# Autodesk Inventor assembly: SPE48V1 Roldana Acrilico
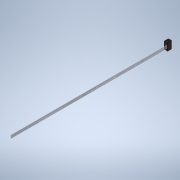
[picture p0: Inventor's stored thumbnail of the model, 180x180]
Saved by Autodesk Inventor 2021.2 (Build 252289000, 289)
## iProperties
Created: 2026-09-01
Part Number: SPE48V1 Roldana Acrilico
Document SubType Name: Assembly
Designer: nelso
Author: nelso
## Documents named in this file (6)
- C:\Users\nelso\Documents\Escritorio\Soporte-Paciente-Espinografia\Workspace\SPE48V1 Roldana Acrilico.iam
- C:\Users\nelso\Documents\Escritorio\Soporte-Paciente-Espinografia\Workspace\SP45V1 Plastico Roldana.ipt
- C:\Users\nelso\Documents\Escritorio\Soporte-Paciente-Espinografia\Workspace\SP46V1 Felpa Roldana.ipt
- C:\Users\nelso\Documents\Escritorio\Soporte-Paciente-Espinografia\Workspace\SP50V1 Acrilico Roldana.ipt
- C:\Users\nelso\Documents\Escritorio\Soporte-Paciente-Espinografia\Workspace\DIN963M3X0.5L10C.ipt
- C:\Users\nelso\Documents\Escritorio\Soporte-Paciente-Espinografia\Workspace\DIN555-5M3X0.5I.ipt
## Components (8 placed, 5 different names)
1. SP45V1 Plastico Roldana:1 — Mate:1, Mate:2, Flush:1, Flush:2, Flush:3, Mate:3, Mate:4, Mate:5, Mate:6, Mate:11, Mate:12
2. SP46V1 Felpa Roldana:1 — Mate:1, Flush:1, Flush:3
3. SP46V1 Felpa Roldana:2 — Mate:2, Flush:2, Mate:3
4. SP50V1 Acrilico Roldana:1 — Mate:4, Mate:5, Mate:6, Mate:7, Flush:4, Mate:8, Flush:5
5. DIN963M3X0.5L10C:1 — Mate:8, Flush:5
6. DIN963M3X0.5L10C:2 — Mate:7, Flush:4
7. DIN555-5M3X0.5I:1 — Mate:12
8. DIN555-5M3X0.5I:2 — Mate:11
## Relationships (15: Mate 10, Flush 5)
- Mate:1: SP45V1 Plastico Roldana:1 ↔ SP46V1 Felpa Roldana:1
- Mate:2: SP45V1 Plastico Roldana:1 ↔ SP46V1 Felpa Roldana:2
- Flush:1: SP45V1 Plastico Roldana:1 ↔ SP46V1 Felpa Roldana:1
- Flush:2: SP45V1 Plastico Roldana:1 ↔ SP46V1 Felpa Roldana:2
- Flush:3: SP45V1 Plastico Roldana:1 ↔ SP46V1 Felpa Roldana:1
- Mate:3: SP45V1 Plastico Roldana:1 ↔ SP46V1 Felpa Roldana:2
- Mate:4: SP45V1 Plastico Roldana:1 ↔ SP50V1 Acrilico Roldana:1
- Mate:5: SP45V1 Plastico Roldana:1 ↔ SP50V1 Acrilico Roldana:1
- Mate:6: SP45V1 Plastico Roldana:1 ↔ SP50V1 Acrilico Roldana:1
- Mate:7: SP50V1 Acrilico Roldana:1 ↔ DIN963M3X0.5L10C:2
- Flush:4: SP50V1 Acrilico Roldana:1 ↔ DIN963M3X0.5L10C:2
- Mate:8: SP50V1 Acrilico Roldana:1 ↔ DIN963M3X0.5L10C:1
- Flush:5: SP50V1 Acrilico Roldana:1 ↔ DIN963M3X0.5L10C:1
- Mate:11: SP45V1 Plastico Roldana:1 ↔ DIN555-5M3X0.5I:2
- Mate:12: SP45V1 Plastico Roldana:1 ↔ DIN555-5M3X0.5I:1
